# Autodesk Inventor assembly: Pedal_Assembly
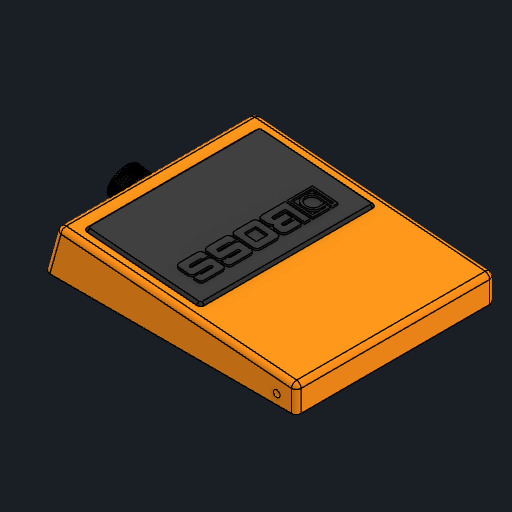
[picture p0: Inventor's stored thumbnail of the model, 512x512]
Saved by Autodesk Inventor 2026.2 (Build 302298000, 298)
## iProperties
Created: 2015-05-06
Part Number: Pedal_Assembly
Document SubType Name: Assembly
Designer: Philip
Author: Philip
## Documents named in this file (4)
- C:\Users\JoshuaEah\Documents\GitHub\Designed-Trinkets\Guitar\Modular Pedalboard\Pedals\Boss Pedal\Pedal_Assembly.iam
- C:\Users\JoshuaEah\Documents\GitHub\Designed-Trinkets\Guitar\Modular Pedalboard\Pedals\Boss Pedal\Pedal.ipt
- C:\Users\JoshuaEah\Documents\GitHub\Designed-Trinkets\Guitar\Modular Pedalboard\Pedals\Boss Pedal\Pad.ipt
- C:\Users\JoshuaEah\Documents\GitHub\Designed-Trinkets\Guitar\Modular Pedalboard\Pedals\Boss Pedal\Knob1.ipt
## Components (3 placed, 3 different names)
1. Pedal:1 — Mate:1, Mate:2, Mate:3, Insert:1
2. Pad:1 — Mate:1, Mate:2, Mate:3
3. Knob1:1 — Insert:1
## Relationships (4: Mate 3, Insert 1)
- Mate:1: Pedal:1 ↔ Pad:1
- Mate:2: Pedal:1 ↔ Pad:1
- Mate:3: Pedal:1 ↔ Pad:1
- Insert:1 (3.175 mm): Pedal:1 ↔ Knob1:1
